# Autodesk Inventor assembly: Flywheel Flipper V1
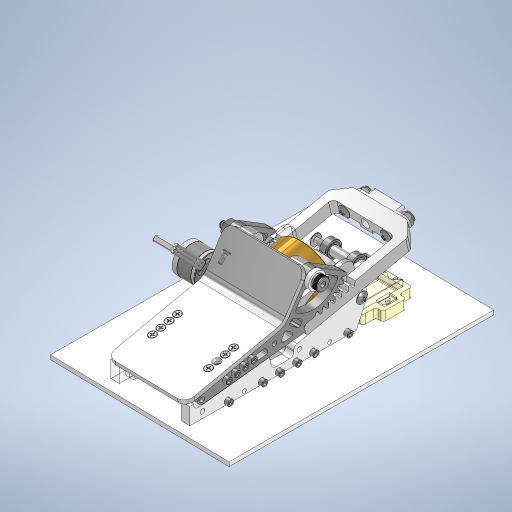
[picture p0: Inventor's stored thumbnail of the model, 512x512]
Saved by Autodesk Inventor 2023.2 (Build 272271000, 271)
## iProperties
Created: 2024-01-10
Part Number: Flywheel Flipper V1
Document SubType Name: Assembly
Designer: Nathan Cai
Mass: 820.137 g
Surface Area: 1996.06 cm^2
Volume: 263.038 cm^3
Density: 3.11794 g/cm^3
Author: Nathan Cai
## Documents named in this file (56)
- E:\Documents\Inventor\Blipper V1\Flywheel Flipper V1.iam
- E:\Documents\Inventor\Blipper V1\Shaft.ipt
- E:\Documents\Inventor\Blipper V1\Bushing.ipt
- E:\Documents\Inventor\Blipper V1\Clutch.ipt
- E:\Documents\Inventor\Blipper V1\Flywheel.ipt
- E:\Documents\Inventor\Blipper V1\Base.ipt
- E:\Documents\Inventor\Blipper V1\Temp - Thrust Bearing.ipt
- E:\Documents\Inventor\Blipper V1\Cup.ipt
- E:\Documents\Inventor\Blipper V1\Uprights.ipt
- E:\Documents\Inventor\Blipper V1\4668K148_Permanently Lubricated Stainless Steel Ball Bearing\4668K148_Permanently Lubricated Stainless Steel Ball Bearing.ipt
- E:\Documents\Inventor\Blipper V1\9731N46_Clamping Two-Piece Shaft Collar\9731N46_Clamping Two-Piece Shaft Collar.ipt
- E:\Documents\Inventor\Blipper V1\BB 13x19x4.ipt
- E:\Documents\Inventor\Blipper V1\Uprights - Cover.ipt
- E:\Documents\Inventor\Blipper V1\Cam - Shell.ipt
- E:\Documents\Inventor\Blipper V1\Cam - Lever.ipt
- E:\Documents\Inventor\Blipper V1\8mm x 16mm Flanged Ball Bearing\8mm x 16mm Flanged Ball Bearing.ipt
- E:\Documents\Inventor\Blipper V1\Part1\Part1.ipt
- E:\Documents\Inventor\Blipper V1\Servo Support.ipt
- E:\Documents\Inventor\Blipper V1\Nut Strip 15x15 - 4-40.ipt
- E:\Documents\Inventor\Blipper V1\Rack.ipt
- E:\Documents\Inventor\Blipper V1\Uprights_MIR.ipt
- E:\Documents\Inventor\Blipper V1\Nut Strip 4x4 - 4-40.ipt
- E:\Documents\Inventor\Blipper V1\Slide.ipt
- E:\Documents\Inventor\Blipper V1\5172T23_Metal Gear - 20 Degree Pressure Angle.ipt
- E:\Documents\Inventor\Blipper V1\Ramp.ipt
- E:\Documents\Inventor\Content Center Files\R2023\en-US\ANSI B18.6.3(12)\ANSI B18.6.3 - 4-40 UNC - 0.3125(15_).ipt
- E:\Documents\Inventor\Blipper V1\Lever.ipt
- E:\Documents\Inventor\Blipper V1\1-4in ID Ball Bearing.ipt
- E:\Documents\Inventor\Blipper V1\Roller.ipt
- E:\Documents\Inventor\Blipper V1\Lever - Clear.ipt
- E:\Documents\Inventor\Blipper V1\Standoff 1in.ipt
- E:\Documents\Inventor\Blipper V1\Pin Slot.ipt
- E:\Documents\Inventor\Content Center Files\R2023\en-US\IFI 100 107(2)\IFI 100_107 - No. 6 - 32 Metal Type.ipt
- E:\Documents\Inventor\Blipper V1\Bushings - Lever.ipt
- E:\Documents\Inventor\Content Center Files\R2023\en-US\ANSI B18.6.3(27)\ANSI B18.6.3 - 6-32 UNC - 0.75(11).ipt
- E:\Documents\Inventor\Content Center Files\R2023\en-US\ANSI B18.6.3(27)\ANSI B18.6.3 - 6-32 UNC - 0.625(11).ipt
- E:\Documents\Inventor\Content Center Files\R2023\en-US\ANSI B18.3(05)\ANSI B18.3 - 4-40 UNC - 0.5(31).ipt
- E:\Documents\Inventor\Content Center Files\R2023\en-US\ANSI B18.3(05)\ANSI B18.3 - 4-40 UNC - 0.625(31).ipt
- E:\Documents\Inventor\Blipper V1\91259A105_Alloy Steel Shoulder Screw\91259A105_Alloy Steel Shoulder Screw.ipt
- E:\Documents\Inventor\Blipper V1\90631A011_Low-Strength Steel Nylon-Insert Locknut\90631A011_Low-Strength Steel Nylon-Insert Locknut.ipt
- E:\Documents\Inventor\Blipper V1\Spacer.ipt
- E:\Documents\Inventor\Blipper V1\Mount PLate.ipt
- E:\Documents\Inventor\Blipper V1\98541A119_External Retaining Ring (1)\98541A119_External Retaining Ring (1).ipt
- E:\Documents\Inventor\Blipper V1\98541A118_External Retaining Ring\98541A118_External Retaining Ring.ipt
- E:\Documents\Inventor\Blipper V1\1561T741_Stacked Wave Disc Spring\1561T741_Stacked Wave Disc Spring.ipt
- E:\Documents\Inventor\Content Center Files\R2023\en-US\ANSI B18.3(05)\ANSI B18.3 - 4-40 UNC - 0.3125(31).ipt
- E:\Documents\Inventor\Content Center Files\R2023\en-US\ASME B18.6.3\ASME B18.6.3 - 4-40.ipt
- E:\Documents\Inventor\Content Center Files\R2023\en-US\ANSI B18.6.3(28)\ANSI B18.6.3 - 6-32 UNC - 0.75(12).ipt
- E:\Documents\Inventor\Blipper V1\Temp - Battery.ipt
- E:\Documents\Inventor\Blipper V1\RDQ ESC32.ipt
- E:\Documents\Inventor\Blipper V1\Aria 35A\Aria 35A.iam
- E:\Documents\Inventor\Blipper V1\22MM\22MM.ipt
- E:\Documents\Inventor\Blipper V1\Side_Plate.ipt
- E:\Documents\Inventor\Blipper V1\Back_Plate.ipt
- E:\Documents\Inventor\Blipper V1\AKK RS2205 2300KV\AKK RS2205 2300KV.iam
- E:\Documents\Inventor\Blipper V1\AKK RS2205 2300KV\AKK RS2205 2300KV - Copy.iam
## Components (111 placed, 55 different names)
1. RDQ ESC32:1
2. RDQ ESC32:2
3. Aria 35A:1 [sub-assembly]
4. 22MM:1 — Mate:736, Flush:69, Mate:773
5. 22MM:2 — Mate:736, Flush:68
6. Side_Plate:1 — Mate:771, Flush:70, Flush:71, Mate:776
7. Side_Plate:2 — Flush:72, Flush:73, Mate:772, Mate:773
8. Temp - Battery:1 — Mate:774
9. Back_Plate:1 — Flush:74, Mate:775, Mate:776
10. AKK RS2205 2300KV:1 [sub-assembly] — Mate:777, Mate:778, Mate:780
11. AKK RS2205 2300KV - Copy:1 [sub-assembly] — Mate:779, Mate:780
12. Shaft:1 — Mate:3, Mate:4, Mate:29, Mate:46, Mate:74, Mate:19, Mate:24, Mate:98, Mate:152, Mate:153, Mate:353, Mate:592, Mate:593, Mate:594, Mate:777, Mate:779
13. Bushing:1 — Mate:3, Mate:4, Mate:5, Mate:7, Mate:34, Mate:116, Mate:117, Mate:590
14. Clutch:1 — Mate:5, Mate:7, Mate:34, Mate:591, Flush:61
15. Flywheel:1 — Mate:19, Mate:46, Mate:89, Mate:90, Mate:97, Mate:150, Mate:154, Flush:61
16. Base:1 — Mate:24, Mate:91, Mate:631, Mate:633, Mate:634, Mate:635, Mate:636, Flush:60, Mate:778
17. Temp - Thrust Bearing:1 — Mate:29, Mate:99, Mate:632
18. Cup:1 — Mate:118, Mate:119, Tangent:5, Angle:2
19. 4668K148_Permanently Lubricated Stainless Steel Ball Bearing:1 — Mate:89, Mate:90, Mate:91
20. 9731N46_Clamping Two-Piece Shaft Collar:1 — Mate:98, Mate:99
21. BB 13x19x4:1 — Mate:116, Mate:117, Mate:118, Mate:119
22. 8mm x 16mm Flanged Ball Bearing:1 — Mate:150, Mate:153, Mate:154
23. 8mm x 16mm Flanged Ball Bearing:2 — Mate:152, Mate:631, Mate:632
24. Cam - Shell:1 — Mate:145, Mate:146, Mate:315, Tangent:4
25. Cam - Lever:1 — Mate:145, Mate:146, Mate:314, Mate:428
26. Part1:1 — Mate:314, Mate:315, Mate:687, Mate:688, Mate:689
27. Servo Support:1 — Mate:686, Mate:687, Mate:688, Mate:689, Flush:65
28. Cross Recessed Flat Countersunk Head Machine Screw - Type I - Inch 4-40 x 5/16:16 — Mate:788
29. Cross Recessed Flat Countersunk Head Machine Screw - Type I - Inch 4-40 x 5/16:15 — Mate:787
30. Cross Recessed Flat Countersunk Head Machine Screw - Type I - Inch 4-40 x 5/16:14 — Mate:786
31. Cross Recessed Flat Countersunk Head Machine Screw - Type I - Inch 4-40 x 5/16:13 — Mate:785
32. Cross Recessed Flat Countersunk Head Machine Screw - Type I - Inch 4-40 x 5/16:12 — Mate:784
33. Cross Recessed Flat Countersunk Head Machine Screw - Type I - Inch 4-40 x 5/16:11 — Mate:783
34. Cross Recessed Flat Countersunk Head Machine Screw - Type I - Inch 4-40 x 5/16:10 — Mate:782
35. Cross Recessed Flat Countersunk Head Machine Screw - Type I - Inch 4-40 x 5/16:1 — Mate:781
36. Prevailing Torque Type Hex Nut - Inch (IFI) No. 6 - 32 Metal Type:2 — Mate:684, Mate:685
37. Cross Recessed Truss Head Machine Screw - Type IA - Inch No. 6 - 32 - 3/4:2 — Mate:680, Mate:681
38. Prevailing Torque Type Hex Nut - Inch (IFI) No. 6 - 32 Metal Type:1 — Mate:682, Mate:683
39. Cross Recessed Truss Head Machine Screw - Type IA - Inch No. 6 - 32 - 3/4:1 — Mate:678, Mate:679
40. Chamfered Bottom Hex Machine Screw Nuts 4-40:1 — Mate:629, Mate:630
41. Cross Recessed Flat Countersunk Head Machine Screw - Type I - Inch 4-40 x 5/16:9 — Mate:628
42. Hexagon Socket Head Cap Screw - Inch No. 4 - 40 UNC - 5/8:7 — Mate:530, Mate:531
43. Hexagon Socket Head Cap Screw - Inch No. 4 - 40 UNC - 5/8:1 — Mate:518, Mate:519
44. Hexagon Socket Head Cap Screw - Inch No. 4 - 40 UNC - 5/8:2 — Mate:520, Mate:521
45. Hexagon Socket Head Cap Screw - Inch No. 4 - 40 UNC - 5/8:3 — Mate:522, Mate:523
46. Hexagon Socket Head Cap Screw - Inch No. 4 - 40 UNC - 5/8:4 — Mate:524, Mate:525
47. Hexagon Socket Head Cap Screw - Inch No. 4 - 40 UNC - 5/8:5 — Mate:526, Mate:527
48. Hexagon Socket Head Cap Screw - Inch No. 4 - 40 UNC - 5/8:6 — Mate:528, Mate:529
49. Hexagon Socket Head Cap Screw - Inch No. 4 - 40 UNC - 5/8:8 — Mate:532, Mate:533
50. Hexagon Socket Head Cap Screw - Inch No. 4 - 40 UNC - 5/8:9 — Mate:534, Mate:535
51. Hexagon Socket Head Cap Screw - Inch No. 4 - 40 UNC - 5/8:10 — Mate:536, Mate:537
52. Hexagon Socket Head Cap Screw - Inch No. 4 - 40 UNC - 5/8:11 — Mate:538, Mate:539
53. Hexagon Socket Head Cap Screw - Inch No. 4 - 40 UNC - 5/8:12 — Mate:540, Mate:541
54. Hexagon Socket Head Cap Screw - Inch No. 4 - 40 UNC - 1/2:8 — Mate:516, Mate:517
55. Hexagon Socket Head Cap Screw - Inch No. 4 - 40 UNC - 1/2:7 — Mate:514, Mate:515
56. Hexagon Socket Head Cap Screw - Inch No. 4 - 40 UNC - 1/2:6 — Mate:512, Mate:513
57. Hexagon Socket Head Cap Screw - Inch No. 4 - 40 UNC - 1/2:5 — Mate:510, Mate:511
58. Hexagon Socket Head Cap Screw - Inch No. 4 - 40 UNC - 1/2:4 — Mate:508, Mate:509
59. Hexagon Socket Head Cap Screw - Inch No. 4 - 40 UNC - 1/2:3 — Mate:506, Mate:507
60. Hexagon Socket Head Cap Screw - Inch No. 4 - 40 UNC - 1/2:2 — Mate:504, Mate:505
61. Hexagon Socket Head Cap Screw - Inch No. 4 - 40 UNC - 1/2:1 — Mate:502, Mate:503
62. Cross Recessed Truss Head Machine Screw - Type I - Inch No. 6 - 32 - 3/4:2 — Mate:460, Mate:461
63. Cross Recessed Truss Head Machine Screw - Type I - Inch No. 6 - 32 - 3/4:3 — Mate:459, Mate:462
64. Cross Recessed Truss Head Machine Screw - Type I - Inch No. 6 - 32 - 5/8:1 — Mate:463, Mate:464
65. Cross Recessed Truss Head Machine Screw - Type I - Inch No. 6 - 32 - 5/8:2 — Mate:465, Mate:466
66. Uprights:1 — Mate:343, Mate:344, Mate:345, Mate:362, Mate:363, Mate:383, Mate:384, Mate:633, Mate:634, Mate:635
67. Uprights - Cover:1 — Mate:347, Mate:348, Mate:352, Mate:354, Flush:51, Flush:52, Mate:380, Mate:381, Mate:382, Mate:431, Mate:432, Mate:455
68. Uprights - Cover:2 — Mate:343, Mate:344, Mate:345, Mate:346, Mate:350, Mate:351, Flush:51, Flush:52, Mate:377, Mate:378, Mate:379, Mate:422, Mate:423, Mate:457
69. Nut Strip 15x15 - 4-40:1 — Mate:347, Mate:348, Mate:352
70. Nut Strip 15x15 - 4-40:2 — Mate:346, Mate:350, Mate:351
71. Rack:1 — Mate:385, Tangent:3, Transitional:1, 60, Mate:353, Mate:354, Rotation/Translation:1, Mate:445, Mate:446, Mate:447, Angle:2, Mate:678, Mate:679, Mate:680, Mate:681, Mate:682, Mate:684
72. Uprights_MIR:1 — Mate:362, Mate:363, Mate:389, Mate:390, Mate:636
73. Nut Strip 4x4 - 4-40:1 — Mate:386, Mate:387, Mate:388
74. Nut Strip 4x4 - 4-40:2 — Mate:392, Mate:393, Mate:394
75. Slide:1 — Mate:377, Mate:378, Mate:379, Mate:459, Mate:462, Mate:530, Mate:531, Mate:532, Mate:533, Mate:534, Mate:535, Mate:536, Mate:537, Mate:538, Mate:539, Mate:540, Mate:541, Mate:557, Flush:63
76. Slide:2 — Mate:380, Mate:381, Mate:382, Mate:460, Mate:461, Mate:518, Mate:519, Mate:520, Mate:521, Mate:522, Mate:523, Mate:524, Mate:525, Mate:526, Mate:527, Mate:528, Mate:529
77. 5172T23_Metal Gear - 20 Degree Pressure Angle:1 — Mate:385, Mate:383, Mate:384, 60, Rotation/Translation:1, Mate:386, Mate:387, Mate:388, Mate:391, Mate:502, Mate:503, Mate:504, Mate:505, Mate:506, Mate:507, Mate:508, Mate:509, Mate:554
78. 5172T23_Metal Gear - 20 Degree Pressure Angle:2 — Mate:389, Mate:390, Mate:391, Mate:392, Mate:393, Mate:394, Mate:396, Flush:55, Mate:397, Mate:510, Mate:511, Mate:512, Mate:513, Mate:514, Mate:515, Mate:516, Mate:517, Mate:551, Mate:552, Mate:555
79. Ramp:1 — Mate:396, Flush:55, Mate:397, Mate:781, Mate:782, Mate:783, Mate:784, Mate:785, Mate:786, Mate:787, Mate:788
80. Lever:1 — Mate:422, Mate:423, Mate:424, Mate:425, Mate:428, Mate:429, Mate:430, Mate:433, Mate:443, Mate:444, Mate:458, Mate:465, Mate:466, Mate:628, Mate:629, Tangent:5
81. Lever - Clear:1 — Mate:431, Mate:432, Mate:433, Mate:434, Mate:435, Mate:456, Mate:463, Mate:464
82. Roller:1 — Mate:429, Mate:430, Tangent:4, Mate:630
83. 1-4in ID Ball Bearing:1 — Mate:424, Mate:425, Tangent:3, Transitional:1
84. 1-4in ID Ball Bearing:2 — Mate:434, Mate:435
85. Standoff 1in:1 — Mate:443, Mate:444
86. Pin Slot:1 — Mate:445, Mate:446, Mate:447, Mate:683, Mate:685
87. Bushings - Lever:1 — Mate:455, Mate:456
88. Bushings - Lever:2 — Mate:457, Mate:458
89. 91259A105_Alloy Steel Shoulder Screw:1 — Mate:551, Mate:552, Mate:553, Mate:556
90. 90631A011_Low-Strength Steel Nylon-Insert Locknut:1 — Mate:553, Mate:554
91. Spacer:1 — Mate:555, Mate:556
92. 98541A119_External Retaining Ring (1):1 — Mate:590, Mate:591
93. 98541A118_External Retaining Ring:1 — Mate:592, Mate:593, Mate:595
94. 1561T741_Stacked Wave Disc Spring:1 — Mate:594, Mate:595
95. Hexagon Socket Head Cap Screw - Inch No. 4 - 40 UNC - 5/16:16 — Mate:768, Mate:769
96. Hexagon Socket Head Cap Screw - Inch No. 4 - 40 UNC - 5/16:15 — Mate:766, Mate:767
97. Hexagon Socket Head Cap Screw - Inch No. 4 - 40 UNC - 5/16:14 — Mate:764, Mate:765
98. Hexagon Socket Head Cap Screw - Inch No. 4 - 40 UNC - 5/16:13 — Mate:762, Mate:763
99. Hexagon Socket Head Cap Screw - Inch No. 4 - 40 UNC - 5/16:12 — Mate:760, Mate:761
100. Hexagon Socket Head Cap Screw - Inch No. 4 - 40 UNC - 5/16:11 — Mate:758, Mate:759
101. Hexagon Socket Head Cap Screw - Inch No. 4 - 40 UNC - 5/16:10 — Mate:756, Mate:757
102. Hexagon Socket Head Cap Screw - Inch No. 4 - 40 UNC - 5/16:9 — Mate:754, Mate:755
103. Hexagon Socket Head Cap Screw - Inch No. 4 - 40 UNC - 5/16:8 — Mate:752, Mate:753
104. Hexagon Socket Head Cap Screw - Inch No. 4 - 40 UNC - 5/16:7 — Mate:750, Mate:751
105. Hexagon Socket Head Cap Screw - Inch No. 4 - 40 UNC - 5/16:6 — Mate:748, Mate:749
106. Hexagon Socket Head Cap Screw - Inch No. 4 - 40 UNC - 5/16:5 — Mate:746, Mate:747
107. Hexagon Socket Head Cap Screw - Inch No. 4 - 40 UNC - 5/16:4 — Mate:744, Mate:745
108. Hexagon Socket Head Cap Screw - Inch No. 4 - 40 UNC - 5/16:3 — Mate:742, Mate:743
109. Hexagon Socket Head Cap Screw - Inch No. 4 - 40 UNC - 5/16:2 — Mate:740, Mate:741
110. Hexagon Socket Head Cap Screw - Inch No. 4 - 40 UNC - 5/16:1 — Mate:738, Mate:739
111. Mount PLate:1 — Mate:557, Flush:62, Mate:677, Mate:686, Flush:63, Flush:65, Flush:68, Flush:69, Mate:738, Mate:739, Mate:740, Mate:741, Mate:742, Mate:743, Mate:744, Mate:745, Mate:746, Mate:747, Mate:748, Mate:749, Mate:750, Mate:751, Mate:752, Mate:753, Mate:754, Mate:755, Mate:756, Mate:757, Mate:758, Mate:759, Mate:760, Mate:761, Mate:762, Mate:763, Mate:764, Mate:765, Mate:766, Mate:767, Mate:768, Mate:769, Mate:771, Flush:70, Flush:71, Flush:72, Flush:73, Mate:772, Mate:774, Flush:74, Mate:775
## Relationships (238: Mate 216, Flush 15, Tangent 3, Angle 2, Transitional 1, RelateRotateTranslate 1)
- Mate:3: Shaft:1 ↔ Bushing:1
- Mate:4: Shaft:1 ↔ Bushing:1
- Mate:5: Bushing:1 ↔ Clutch:1
- Mate:7: Bushing:1 ↔ Clutch:1
- Mate:19: Shaft:1 ↔ Flywheel:1
- Mate:24: Shaft:1 ↔ Base:1
- Mate:29: Shaft:1 ↔ Temp - Thrust Bearing:1
- Mate:34: Bushing:1 ↔ Clutch:1
- Mate:46: Shaft:1 ↔ Flywheel:1
- Mate:74: Shaft:1
- Mate:89: Flywheel:1 ↔ 4668K148_Permanently Lubricated Stainless Steel Ball Bearing:1
- Mate:90: Flywheel:1 ↔ 4668K148_Permanently Lubricated Stainless Steel Ball Bearing:1
- Mate:91: Base:1 ↔ 4668K148_Permanently Lubricated Stainless Steel Ball Bearing:1
- Mate:97: Flywheel:1
- Mate:98: Shaft:1 ↔ 9731N46_Clamping Two-Piece Shaft Collar:1
- Mate:99: Temp - Thrust Bearing:1 ↔ 9731N46_Clamping Two-Piece Shaft Collar:1
- Mate:116: Bushing:1 ↔ BB 13x19x4:1
- Mate:117: Bushing:1 ↔ BB 13x19x4:1
- Mate:118: Cup:1 ↔ BB 13x19x4:1
- Mate:119: Cup:1 ↔ BB 13x19x4:1
- Mate:145: Cam - Shell:1 ↔ Cam - Lever:1
- Mate:146: Cam - Shell:1 ↔ Cam - Lever:1
- Mate:150: Flywheel:1 ↔ 8mm x 16mm Flanged Ball Bearing:1
- Mate:152: Shaft:1 ↔ 8mm x 16mm Flanged Ball Bearing:2
- Mate:153: Shaft:1 ↔ 8mm x 16mm Flanged Ball Bearing:1
- Mate:154: Flywheel:1 ↔ 8mm x 16mm Flanged Ball Bearing:1
- Mate:314: Cam - Lever:1 ↔ Part1:1
- Mate:315: Cam - Shell:1 ↔ Part1:1
- Mate:343: Uprights:1 ↔ Uprights - Cover:2
- Mate:344: Uprights:1 ↔ Uprights - Cover:2
- Mate:345: Uprights:1 ↔ Uprights - Cover:2
- Mate:346: Uprights - Cover:2 ↔ Nut Strip 15x15 - 4-40:2
- Mate:347: Uprights - Cover:1 ↔ Nut Strip 15x15 - 4-40:1
- Mate:348: Uprights - Cover:1 ↔ Nut Strip 15x15 - 4-40:1
- Mate:350: Uprights - Cover:2 ↔ Nut Strip 15x15 - 4-40:2
- Mate:351: Uprights - Cover:2 ↔ Nut Strip 15x15 - 4-40:2
- Mate:352: Uprights - Cover:1 ↔ Nut Strip 15x15 - 4-40:1
- Mate:385: Rack:1 ↔ 5172T23_Metal Gear - 20 Degree Pressure Angle:1
- Tangent:3: Rack:1 ↔ 1-4in ID Ball Bearing:1
- Transitional:1: Rack:1 ↔ 1-4in ID Ball Bearing:1
- 60 [Angle] (0 deg): Rack:1 ↔ 5172T23_Metal Gear - 20 Degree Pressure Angle:1
- Mate:353: Shaft:1 ↔ Rack:1
- Mate:354: Uprights - Cover:1 ↔ Rack:1
- Flush:51: Uprights - Cover:1 ↔ Uprights - Cover:2
- Flush:52: Uprights - Cover:1 ↔ Uprights - Cover:2
- Mate:362: Uprights:1 ↔ Uprights_MIR:1
- Mate:363: Uprights:1 ↔ Uprights_MIR:1
- Mate:377: Uprights - Cover:2 ↔ Slide:1
- Mate:378: Uprights - Cover:2 ↔ Slide:1
- Mate:379: Uprights - Cover:2 ↔ Slide:1
- Mate:380: Uprights - Cover:1 ↔ Slide:2
- Mate:381: Uprights - Cover:1 ↔ Slide:2
- Mate:382: Uprights - Cover:1 ↔ Slide:2
- Mate:383: Uprights:1 ↔ 5172T23_Metal Gear - 20 Degree Pressure Angle:1
- Mate:384: Uprights:1 ↔ 5172T23_Metal Gear - 20 Degree Pressure Angle:1
- Rotation/Translation:1 [RelateRotateTranslate] (159.5933 mm): Rack:1 ↔ 5172T23_Metal Gear - 20 Degree Pressure Angle:1
- Mate:386: Nut Strip 4x4 - 4-40:1 ↔ 5172T23_Metal Gear - 20 Degree Pressure Angle:1
- Mate:387: Nut Strip 4x4 - 4-40:1 ↔ 5172T23_Metal Gear - 20 Degree Pressure Angle:1
- Mate:388: Nut Strip 4x4 - 4-40:1 ↔ 5172T23_Metal Gear - 20 Degree Pressure Angle:1
- Mate:389: Uprights_MIR:1 ↔ 5172T23_Metal Gear - 20 Degree Pressure Angle:2
- Mate:390: Uprights_MIR:1 ↔ 5172T23_Metal Gear - 20 Degree Pressure Angle:2
- Mate:391: 5172T23_Metal Gear - 20 Degree Pressure Angle:1 ↔ 5172T23_Metal Gear - 20 Degree Pressure Angle:2
- Mate:392: Nut Strip 4x4 - 4-40:2 ↔ 5172T23_Metal Gear - 20 Degree Pressure Angle:2
- Mate:393: Nut Strip 4x4 - 4-40:2 ↔ 5172T23_Metal Gear - 20 Degree Pressure Angle:2
- Mate:394: Nut Strip 4x4 - 4-40:2 ↔ 5172T23_Metal Gear - 20 Degree Pressure Angle:2
- Mate:396: 5172T23_Metal Gear - 20 Degree Pressure Angle:2 ↔ Ramp:1
- Flush:55: 5172T23_Metal Gear - 20 Degree Pressure Angle:2 ↔ Ramp:1
- Mate:397: 5172T23_Metal Gear - 20 Degree Pressure Angle:2 ↔ Ramp:1
- Mate:422: Uprights - Cover:2 ↔ Lever:1
- Mate:423: Uprights - Cover:2 ↔ Lever:1
- Mate:424: Lever:1 ↔ 1-4in ID Ball Bearing:1
- Mate:425 (0.7937 mm): Lever:1 ↔ 1-4in ID Ball Bearing:1
- Mate:428: Cam - Lever:1 ↔ Lever:1
- Mate:429: Lever:1 ↔ Roller:1
- Mate:430: Lever:1 ↔ Roller:1
- Tangent:4: Cam - Shell:1 ↔ Roller:1
- Mate:431: Uprights - Cover:1 ↔ Lever - Clear:1
- Mate:432: Uprights - Cover:1 ↔ Lever - Clear:1
- Mate:433: Lever:1 ↔ Lever - Clear:1
- Mate:434 (0.7937 mm): Lever - Clear:1 ↔ 1-4in ID Ball Bearing:2
- Mate:435: Lever - Clear:1 ↔ 1-4in ID Ball Bearing:2
- Mate:443: Lever:1 ↔ Standoff 1in:1
- Mate:444: Lever:1 ↔ Standoff 1in:1
- Mate:445: Rack:1 ↔ Pin Slot:1
- Mate:446: Rack:1 ↔ Pin Slot:1
- Mate:447: Rack:1 ↔ Pin Slot:1
- Mate:455: Uprights - Cover:1 ↔ Bushings - Lever:1
- Mate:456: Lever - Clear:1 ↔ Bushings - Lever:1
- Mate:457: Uprights - Cover:2 ↔ Bushings - Lever:2
- Mate:458: Lever:1 ↔ Bushings - Lever:2
- Mate:459: Cross Recessed Truss Head Machine Screw - Type I - Inch No. 6 - 32 - 3/4:3 ↔ Slide:1
- Mate:460: Cross Recessed Truss Head Machine Screw - Type I - Inch No. 6 - 32 - 3/4:2 ↔ Slide:2
- Mate:461: Cross Recessed Truss Head Machine Screw - Type I - Inch No. 6 - 32 - 3/4:2 ↔ Slide:2
- Mate:462: Cross Recessed Truss Head Machine Screw - Type I - Inch No. 6 - 32 - 3/4:3 ↔ Slide:1
- Mate:463: Cross Recessed Truss Head Machine Screw - Type I - Inch No. 6 - 32 - 5/8:1 ↔ Lever - Clear:1
- Mate:464: Cross Recessed Truss Head Machine Screw - Type I - Inch No. 6 - 32 - 5/8:1 ↔ Lever - Clear:1
- Mate:465: Cross Recessed Truss Head Machine Screw - Type I - Inch No. 6 - 32 - 5/8:2 ↔ Lever:1
- Mate:466: Cross Recessed Truss Head Machine Screw - Type I - Inch No. 6 - 32 - 5/8:2 ↔ Lever:1
- Mate:502: Hexagon Socket Head Cap Screw - Inch No. 4 - 40 UNC - 1/2:1 ↔ 5172T23_Metal Gear - 20 Degree Pressure Angle:1
- Mate:503: Hexagon Socket Head Cap Screw - Inch No. 4 - 40 UNC - 1/2:1 ↔ 5172T23_Metal Gear - 20 Degree Pressure Angle:1
- Mate:504: Hexagon Socket Head Cap Screw - Inch No. 4 - 40 UNC - 1/2:2 ↔ 5172T23_Metal Gear - 20 Degree Pressure Angle:1
- Mate:505: Hexagon Socket Head Cap Screw - Inch No. 4 - 40 UNC - 1/2:2 ↔ 5172T23_Metal Gear - 20 Degree Pressure Angle:1
- Mate:506: Hexagon Socket Head Cap Screw - Inch No. 4 - 40 UNC - 1/2:3 ↔ 5172T23_Metal Gear - 20 Degree Pressure Angle:1
- Mate:507: Hexagon Socket Head Cap Screw - Inch No. 4 - 40 UNC - 1/2:3 ↔ 5172T23_Metal Gear - 20 Degree Pressure Angle:1
- Mate:508: Hexagon Socket Head Cap Screw - Inch No. 4 - 40 UNC - 1/2:4 ↔ 5172T23_Metal Gear - 20 Degree Pressure Angle:1
- Mate:509: Hexagon Socket Head Cap Screw - Inch No. 4 - 40 UNC - 1/2:4 ↔ 5172T23_Metal Gear - 20 Degree Pressure Angle:1
- Mate:510: Hexagon Socket Head Cap Screw - Inch No. 4 - 40 UNC - 1/2:5 ↔ 5172T23_Metal Gear - 20 Degree Pressure Angle:2
- Mate:511: Hexagon Socket Head Cap Screw - Inch No. 4 - 40 UNC - 1/2:5 ↔ 5172T23_Metal Gear - 20 Degree Pressure Angle:2
- Mate:512: Hexagon Socket Head Cap Screw - Inch No. 4 - 40 UNC - 1/2:6 ↔ 5172T23_Metal Gear - 20 Degree Pressure Angle:2
- Mate:513: Hexagon Socket Head Cap Screw - Inch No. 4 - 40 UNC - 1/2:6 ↔ 5172T23_Metal Gear - 20 Degree Pressure Angle:2
- Mate:514: Hexagon Socket Head Cap Screw - Inch No. 4 - 40 UNC - 1/2:7 ↔ 5172T23_Metal Gear - 20 Degree Pressure Angle:2
- Mate:515: Hexagon Socket Head Cap Screw - Inch No. 4 - 40 UNC - 1/2:7 ↔ 5172T23_Metal Gear - 20 Degree Pressure Angle:2
- Mate:516: Hexagon Socket Head Cap Screw - Inch No. 4 - 40 UNC - 1/2:8 ↔ 5172T23_Metal Gear - 20 Degree Pressure Angle:2
- Mate:517: Hexagon Socket Head Cap Screw - Inch No. 4 - 40 UNC - 1/2:8 ↔ 5172T23_Metal Gear - 20 Degree Pressure Angle:2
- Mate:518: Hexagon Socket Head Cap Screw - Inch No. 4 - 40 UNC - 5/8:1 ↔ Slide:2
- Mate:519: Hexagon Socket Head Cap Screw - Inch No. 4 - 40 UNC - 5/8:1 ↔ Slide:2
- Mate:520: Hexagon Socket Head Cap Screw - Inch No. 4 - 40 UNC - 5/8:2 ↔ Slide:2
- Mate:521: Hexagon Socket Head Cap Screw - Inch No. 4 - 40 UNC - 5/8:2 ↔ Slide:2
- Mate:522: Hexagon Socket Head Cap Screw - Inch No. 4 - 40 UNC - 5/8:3 ↔ Slide:2
- Mate:523: Hexagon Socket Head Cap Screw - Inch No. 4 - 40 UNC - 5/8:3 ↔ Slide:2
- Mate:524: Hexagon Socket Head Cap Screw - Inch No. 4 - 40 UNC - 5/8:4 ↔ Slide:2
- Mate:525: Hexagon Socket Head Cap Screw - Inch No. 4 - 40 UNC - 5/8:4 ↔ Slide:2
- Mate:526: Hexagon Socket Head Cap Screw - Inch No. 4 - 40 UNC - 5/8:5 ↔ Slide:2
- Mate:527: Hexagon Socket Head Cap Screw - Inch No. 4 - 40 UNC - 5/8:5 ↔ Slide:2
- Mate:528: Hexagon Socket Head Cap Screw - Inch No. 4 - 40 UNC - 5/8:6 ↔ Slide:2
- Mate:529: Hexagon Socket Head Cap Screw - Inch No. 4 - 40 UNC - 5/8:6 ↔ Slide:2
- Mate:530: Hexagon Socket Head Cap Screw - Inch No. 4 - 40 UNC - 5/8:7 ↔ Slide:1
- Mate:531: Hexagon Socket Head Cap Screw - Inch No. 4 - 40 UNC - 5/8:7 ↔ Slide:1
- Mate:532: Hexagon Socket Head Cap Screw - Inch No. 4 - 40 UNC - 5/8:8 ↔ Slide:1
- Mate:533: Hexagon Socket Head Cap Screw - Inch No. 4 - 40 UNC - 5/8:8 ↔ Slide:1
- Mate:534: Hexagon Socket Head Cap Screw - Inch No. 4 - 40 UNC - 5/8:9 ↔ Slide:1
- Mate:535: Hexagon Socket Head Cap Screw - Inch No. 4 - 40 UNC - 5/8:9 ↔ Slide:1
- Mate:536: Hexagon Socket Head Cap Screw - Inch No. 4 - 40 UNC - 5/8:10 ↔ Slide:1
- Mate:537: Hexagon Socket Head Cap Screw - Inch No. 4 - 40 UNC - 5/8:10 ↔ Slide:1
- Mate:538: Hexagon Socket Head Cap Screw - Inch No. 4 - 40 UNC - 5/8:11 ↔ Slide:1
- Mate:539: Hexagon Socket Head Cap Screw - Inch No. 4 - 40 UNC - 5/8:11 ↔ Slide:1
- Mate:540: Hexagon Socket Head Cap Screw - Inch No. 4 - 40 UNC - 5/8:12 ↔ Slide:1
- Mate:541: Hexagon Socket Head Cap Screw - Inch No. 4 - 40 UNC - 5/8:12 ↔ Slide:1
- Mate:551: 5172T23_Metal Gear - 20 Degree Pressure Angle:2 ↔ 91259A105_Alloy Steel Shoulder Screw:1
- Mate:552 (3.175 mm): 5172T23_Metal Gear - 20 Degree Pressure Angle:2 ↔ 91259A105_Alloy Steel Shoulder Screw:1
- Mate:553: 91259A105_Alloy Steel Shoulder Screw:1 ↔ 90631A011_Low-Strength Steel Nylon-Insert Locknut:1
- Mate:554: 5172T23_Metal Gear - 20 Degree Pressure Angle:1 ↔ 90631A011_Low-Strength Steel Nylon-Insert Locknut:1
- Mate:555: 5172T23_Metal Gear - 20 Degree Pressure Angle:2 ↔ Spacer:1
- Mate:556: 91259A105_Alloy Steel Shoulder Screw:1 ↔ Spacer:1
- Mate:557: Slide:1 ↔ Mount PLate:1
- Mate:590: Bushing:1 ↔ 98541A119_External Retaining Ring (1):1
- Mate:591: Clutch:1 ↔ 98541A119_External Retaining Ring (1):1
- Mate:592: Shaft:1 ↔ 98541A118_External Retaining Ring:1
- Mate:593: Shaft:1 ↔ 98541A118_External Retaining Ring:1
- Mate:594: Shaft:1 ↔ 1561T741_Stacked Wave Disc Spring:1
- Mate:595: 98541A118_External Retaining Ring:1 ↔ 1561T741_Stacked Wave Disc Spring:1
- Mate:628: Cross Recessed Flat Countersunk Head Machine Screw - Type I - Inch 4-40 x 5/16:9 ↔ Lever:1
- Mate:629: Chamfered Bottom Hex Machine Screw Nuts 4-40:1 ↔ Lever:1
- Mate:630: Chamfered Bottom Hex Machine Screw Nuts 4-40:1 ↔ Roller:1
- Mate:631: Base:1 ↔ 8mm x 16mm Flanged Ball Bearing:2
- Mate:632: Temp - Thrust Bearing:1 ↔ 8mm x 16mm Flanged Ball Bearing:2
- Mate:633: Base:1 ↔ Uprights:1
- Mate:634: Base:1 ↔ Uprights:1
- Mate:635: Base:1 ↔ Uprights:1
- Mate:636: Base:1 ↔ Uprights_MIR:1
- Flush:60: Base:1
- Tangent:5: Cup:1 ↔ Lever:1
- Flush:61 (-1.5 mm): Clutch:1 ↔ Flywheel:1
- Flush:62: Mount PLate:1
- Angle:2 (0 deg): Cup:1 ↔ Rack:1
- Mate:677: Mount PLate:1
- Mate:678: Cross Recessed Truss Head Machine Screw - Type IA - Inch No. 6 - 32 - 3/4:1 ↔ Rack:1
- Mate:679: Cross Recessed Truss Head Machine Screw - Type IA - Inch No. 6 - 32 - 3/4:1 ↔ Rack:1
- Mate:680: Cross Recessed Truss Head Machine Screw - Type IA - Inch No. 6 - 32 - 3/4:2 ↔ Rack:1
- Mate:681: Cross Recessed Truss Head Machine Screw - Type IA - Inch No. 6 - 32 - 3/4:2 ↔ Rack:1
- Mate:682: Prevailing Torque Type Hex Nut - Inch (IFI) No. 6 - 32 Metal Type:1 ↔ Rack:1
- Mate:683: Prevailing Torque Type Hex Nut - Inch (IFI) No. 6 - 32 Metal Type:1 ↔ Pin Slot:1
- Mate:684: Prevailing Torque Type Hex Nut - Inch (IFI) No. 6 - 32 Metal Type:2 ↔ Rack:1
- Mate:685: Prevailing Torque Type Hex Nut - Inch (IFI) No. 6 - 32 Metal Type:2 ↔ Pin Slot:1
- Mate:686: Servo Support:1 ↔ Mount PLate:1
- Mate:687: Part1:1 ↔ Servo Support:1
- Mate:688: Part1:1 ↔ Servo Support:1
- Mate:689: Part1:1 ↔ Servo Support:1
- Flush:63 (7.9375 mm): Slide:1 ↔ Mount PLate:1
- Flush:65 (19.05 mm): Servo Support:1 ↔ Mount PLate:1
- Mate:736: 22MM:1 ↔ 22MM:2
- Flush:68: 22MM:2 ↔ Mount PLate:1
- Flush:69: 22MM:1 ↔ Mount PLate:1
- Mate:738: Hexagon Socket Head Cap Screw - Inch No. 4 - 40 UNC - 5/16:1 ↔ Mount PLate:1
- Mate:739: Hexagon Socket Head Cap Screw - Inch No. 4 - 40 UNC - 5/16:1 ↔ Mount PLate:1
- Mate:740: Hexagon Socket Head Cap Screw - Inch No. 4 - 40 UNC - 5/16:2 ↔ Mount PLate:1
- Mate:741: Hexagon Socket Head Cap Screw - Inch No. 4 - 40 UNC - 5/16:2 ↔ Mount PLate:1
- Mate:742: Hexagon Socket Head Cap Screw - Inch No. 4 - 40 UNC - 5/16:3 ↔ Mount PLate:1
- Mate:743: Hexagon Socket Head Cap Screw - Inch No. 4 - 40 UNC - 5/16:3 ↔ Mount PLate:1
- Mate:744: Hexagon Socket Head Cap Screw - Inch No. 4 - 40 UNC - 5/16:4 ↔ Mount PLate:1
- Mate:745: Hexagon Socket Head Cap Screw - Inch No. 4 - 40 UNC - 5/16:4 ↔ Mount PLate:1
- Mate:746: Hexagon Socket Head Cap Screw - Inch No. 4 - 40 UNC - 5/16:5 ↔ Mount PLate:1
- Mate:747: Hexagon Socket Head Cap Screw - Inch No. 4 - 40 UNC - 5/16:5 ↔ Mount PLate:1
- Mate:748: Hexagon Socket Head Cap Screw - Inch No. 4 - 40 UNC - 5/16:6 ↔ Mount PLate:1
- Mate:749: Hexagon Socket Head Cap Screw - Inch No. 4 - 40 UNC - 5/16:6 ↔ Mount PLate:1
- Mate:750: Hexagon Socket Head Cap Screw - Inch No. 4 - 40 UNC - 5/16:7 ↔ Mount PLate:1
- Mate:751: Hexagon Socket Head Cap Screw - Inch No. 4 - 40 UNC - 5/16:7 ↔ Mount PLate:1
- Mate:752: Hexagon Socket Head Cap Screw - Inch No. 4 - 40 UNC - 5/16:8 ↔ Mount PLate:1
- Mate:753: Hexagon Socket Head Cap Screw - Inch No. 4 - 40 UNC - 5/16:8 ↔ Mount PLate:1
- Mate:754: Hexagon Socket Head Cap Screw - Inch No. 4 - 40 UNC - 5/16:9 ↔ Mount PLate:1
- Mate:755: Hexagon Socket Head Cap Screw - Inch No. 4 - 40 UNC - 5/16:9 ↔ Mount PLate:1
- Mate:756: Hexagon Socket Head Cap Screw - Inch No. 4 - 40 UNC - 5/16:10 ↔ Mount PLate:1
- Mate:757: Hexagon Socket Head Cap Screw - Inch No. 4 - 40 UNC - 5/16:10 ↔ Mount PLate:1
- Mate:758: Hexagon Socket Head Cap Screw - Inch No. 4 - 40 UNC - 5/16:11 ↔ Mount PLate:1
- Mate:759: Hexagon Socket Head Cap Screw - Inch No. 4 - 40 UNC - 5/16:11 ↔ Mount PLate:1
- Mate:760: Hexagon Socket Head Cap Screw - Inch No. 4 - 40 UNC - 5/16:12 ↔ Mount PLate:1
- Mate:761: Hexagon Socket Head Cap Screw - Inch No. 4 - 40 UNC - 5/16:12 ↔ Mount PLate:1
- Mate:762: Hexagon Socket Head Cap Screw - Inch No. 4 - 40 UNC - 5/16:13 ↔ Mount PLate:1
- Mate:763: Hexagon Socket Head Cap Screw - Inch No. 4 - 40 UNC - 5/16:13 ↔ Mount PLate:1
- Mate:764: Hexagon Socket Head Cap Screw - Inch No. 4 - 40 UNC - 5/16:14 ↔ Mount PLate:1
- Mate:765: Hexagon Socket Head Cap Screw - Inch No. 4 - 40 UNC - 5/16:14 ↔ Mount PLate:1
- Mate:766: Hexagon Socket Head Cap Screw - Inch No. 4 - 40 UNC - 5/16:15 ↔ Mount PLate:1
- Mate:767: Hexagon Socket Head Cap Screw - Inch No. 4 - 40 UNC - 5/16:15 ↔ Mount PLate:1
- Mate:768: Hexagon Socket Head Cap Screw - Inch No. 4 - 40 UNC - 5/16:16 ↔ Mount PLate:1
- Mate:769: Hexagon Socket Head Cap Screw - Inch No. 4 - 40 UNC - 5/16:16 ↔ Mount PLate:1
- Mate:771: Side_Plate:1 ↔ Mount PLate:1
- Flush:70: Side_Plate:1 ↔ Mount PLate:1
- Flush:71: Side_Plate:1 ↔ Mount PLate:1
- Flush:72: Side_Plate:2 ↔ Mount PLate:1
- Flush:73: Side_Plate:2 ↔ Mount PLate:1
- Mate:772: Side_Plate:2 ↔ Mount PLate:1
- Mate:773: 22MM:1 ↔ Side_Plate:2
- Mate:774: Temp - Battery:1 ↔ Mount PLate:1
- Flush:74: Back_Plate:1 ↔ Mount PLate:1
- Mate:775: Back_Plate:1 ↔ Mount PLate:1
- Mate:776: Side_Plate:1 ↔ Back_Plate:1
- Mate:777: AKK RS2205 2300KV:1 ↔ Shaft:1
- Mate:778: AKK RS2205 2300KV:1 ↔ Base:1
- Mate:779: AKK RS2205 2300KV - Copy:1 ↔ Shaft:1
- Mate:780 (0.5 mm): AKK RS2205 2300KV:1 ↔ AKK RS2205 2300KV - Copy:1
- Mate:781: Cross Recessed Flat Countersunk Head Machine Screw - Type I - Inch 4-40 x 5/16:1 ↔ Ramp:1
- Mate:782: Cross Recessed Flat Countersunk Head Machine Screw - Type I - Inch 4-40 x 5/16:10 ↔ Ramp:1
- Mate:783: Cross Recessed Flat Countersunk Head Machine Screw - Type I - Inch 4-40 x 5/16:11 ↔ Ramp:1
- Mate:784: Cross Recessed Flat Countersunk Head Machine Screw - Type I - Inch 4-40 x 5/16:12 ↔ Ramp:1
- Mate:785: Cross Recessed Flat Countersunk Head Machine Screw - Type I - Inch 4-40 x 5/16:13 ↔ Ramp:1
- Mate:786: Cross Recessed Flat Countersunk Head Machine Screw - Type I - Inch 4-40 x 5/16:14 ↔ Ramp:1
- Mate:787: Cross Recessed Flat Countersunk Head Machine Screw - Type I - Inch 4-40 x 5/16:15 ↔ Ramp:1
- Mate:788: Cross Recessed Flat Countersunk Head Machine Screw - Type I - Inch 4-40 x 5/16:16 ↔ Ramp:1
